# Autodesk Inventor assembly: IntakeAssembly-ver1-1111-2020
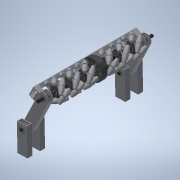
[picture p0: Inventor's stored thumbnail of the model, 180x180]
Saved by Autodesk Inventor 2021 (Build 250183000, 183)
## iProperties
Created: 2020-01-11
Part Number: IntakeAssembly-ver1-1111-2020
Document SubType Name: Assembly
Designer: Power Hawks CADD
Author: Power Hawks CADD
## Documents named in this file (14)
- E:\PHRC CADD 2021\PHRC CADD\2020 Infinite Recharge\Intake\Assemblies\IntakeAssembly-ver1-1111-2020.iam
- E:\PHRC CADD 2021\PHRC CADD\2020 Infinite Recharge\Intake\Parts\0.5inThunderHexShaft-1111-2020.ipt
- E:\PHRC CADD 2021\PHRC CADD\2020 Infinite Recharge\Intake\Parts\Mechanum Wheel.iam
- E:\PHRC CADD 2021\PHRC CADD\2020 Infinite Recharge\Intake\Parts\0.5inAcetalSpacer-1111-2020.ipt
- E:\PHRC CADD 2021\PHRC CADD\Resources\VEXpro Resources\Wheels\4 inch\4IN-CompliantWheel-500Hex.iam
- E:\PHRC CADD 2021\PHRC CADD\Resources\VEXpro Resources\Spacers\0.5inAcetalSpace(0.5inHex)-1111-2016.ipt
- E:\PHRC CADD 2021\PHRC CADD\Resources\VEXpro Resources\Wheels\Mecanum Wheels\4_Mecanum_Wheel_Left_217-3644.iam
- E:\PHRC CADD 2021\PHRC CADD\2020 Infinite Recharge\Intake\Parts\WristBarr.ver1-1111-2020.ipt
- E:\PHRC CADD 2021\PHRC CADD\Resources\VEXpro Resources\Bearings\0.5inHexFlangedBearing(1.125inx0.313in)-1111-2016.ipt
- E:\PHRC CADD 2021\PHRC CADD\2020 Infinite Recharge\Intake\Parts\1x2AluminumSpacer.ver1-1111-2020.ipt
- E:\PHRC CADD 2021\PHRC CADD\2020 Infinite Recharge\Intake\Parts\OverheadSupportBar.ver1-1111-2020.ipt
- E:\PHRC CADD 2021\PHRC CADD\2020 Infinite Recharge\Intake\Parts\WristFulcrum.ver-1111-2020.ipt
- E:\PHRC CADD 2021\PHRC CADD\2020 Infinite Recharge\Intake\Parts\0.5inThunderHexShaft4in-1111-2020.ipt
- E:\PHRC CADD 2021\PHRC CADD\Resources\VEXpro Resources\Spacers\0.125inAcetalSpacer(0.5inHex)-1111-2016.ipt
## Components (47 placed, 13 different names)
1. 0.5inThunderHexShaft-1111-2020:1 — Cylindrical:1, Cylindrical:2, Cylindrical:3, Cylindrical:4, Cylindrical:5, Cylindrical:6, Cylindrical:7, Cylindrical:8, Cylindrical:10, Cylindrical:11, Cylindrical:12, Cylindrical:13, Cylindrical:14, Cylindrical:15, Cylindrical:22, Cylindrical:25, Flush:8
2. Mechanum Wheel:1 [sub-assembly] — Cylindrical:3, Mate:6, Mate:14
3. Mechanum Wheel:2 [sub-assembly] — Cylindrical:2, Mate:8, Mate:9
4. Mechanum Wheel:3 [sub-assembly] — Cylindrical:7, Mate:4, Mate:5
5. Mechanum Wheel:4 [sub-assembly] — Cylindrical:5, Mate:2, Mate:3
6. 0.5inAcetalSpacer-1111-2020:1 — Cylindrical:1, Mate:5, Mate:6
7. 0.5inAcetalSpacer-1111-2020:2 — Cylindrical:4, Mate:1, Mate:2
8. 0.5inAcetalSpacer-1111-2020:3 — Cylindrical:6, Mate:3, Mate:4
9. 4IN-CompliantWheel-500Hex:1 [sub-assembly] — Cylindrical:8, Mate:1, Cylindrical:9, Mate:7
10. 0.5inAcetalSpace(0.5inHex)-1111-2016:1 — Cylindrical:9, Mate:7, Mate:8
11. 0.5inAcetalSpace(0.5inHex)-1111-2016:2 — Cylindrical:10, Mate:9, Mate:10
12. 0.5inAcetalSpace(0.5inHex)-1111-2016:3 — Cylindrical:14, Mate:13, Mate:30
13. 0.5inAcetalSpace(0.5inHex)-1111-2016:4 — Cylindrical:12, Mate:11, Mate:12
14. 4_Mecanum_Wheel_Left_217-3644:1 [sub-assembly] — Cylindrical:13, Mate:12, Mate:13
15. 4_Mecanum_Wheel_Left_217-3644:2 [sub-assembly] — Cylindrical:11, Mate:10, Mate:11
16. 0.5inAcetalSpace(0.5inHex)-1111-2016:5 — Cylindrical:15, Mate:14, Mate:31
17. WristBarr.ver1-1111-2020:1 — Cylindrical:20, Mate:18, Cylindrical:21, Mate:19, Flush:2, Mate:25, Flush:3, Mate:26, Cylindrical:26, Mate:29, Rigid:1
18. WristBarr.ver1-1111-2020:2 — Cylindrical:23, Cylindrical:24, Mate:22, Mate:23, Flush:2, Mate:28, Flush:6, Rigid:2, Rigid:3, Flush:8
19. 0.5inHexFlangedBearing(1.125inx0.313in)-1111-2016:1 — Cylindrical:24, Mate:22
20. 0.5inHexFlangedBearing(1.125inx0.313in)-1111-2016:2 — Cylindrical:23, Mate:23, Cylindrical:25, Mate:30
21. 0.5inHexFlangedBearing(1.125inx0.313in)-1111-2016:4 — Cylindrical:20, Mate:18
22. 0.5inHexFlangedBearing(1.125inx0.313in)-1111-2016:8 — Cylindrical:21, Mate:19, Cylindrical:22, Mate:31
23. OverheadSupportBar.ver1-1111-2020:1 — Mate:27, Flush:4, Flush:5, Flush:7
24. 1x2AluminumSpacer.ver1-1111-2020:1 — Mate:25, Flush:3, Mate:26, Mate:27, Flush:4, Flush:5
25. 1x2AluminumSpacer.ver1-1111-2020:2 — Mate:28, Flush:6, Flush:7
26. 0.5inHexFlangedBearing(1.125inx0.313in)-1111-2016:9 — Rigid:2, Mate:36
27. 0.5inHexFlangedBearing(1.125inx0.313in)-1111-2016:10 — Cylindrical:26, Mate:29, Cylindrical:28, Mate:32
28. 0.5inHexFlangedBearing(1.125inx0.313in)-1111-2016:11 — Rigid:3, Cylindrical:27, Mate:37
29. 0.5inHexFlangedBearing(1.125inx0.313in)-1111-2016:12 — Rigid:1, Mate:34
30. WristFulcrum.ver-1111-2020:1 — Rotational:1, Rotational:2, Flush:9, Flush:10
31. WristFulcrum.ver-1111-2020:2 — Rotational:3, Rotational:4, Flush:9
32. WristFulcrum.ver-1111-2020:3 — Rotational:5, Rotational:6, Flush:10, Flush:11
33. WristFulcrum.ver-1111-2020:4 — Rotational:7, Rotational:8, Flush:11
34. 0.5inHexFlangedBearing(1.125inx0.313in)-1111-2016:13 — Rotational:1, Cylindrical:30, Mate:35
35. 0.5inHexFlangedBearing(1.125inx0.313in)-1111-2016:14 — Rotational:4, Cylindrical:29, Mate:33
36. 0.5inHexFlangedBearing(1.125inx0.313in)-1111-2016:15 — Rotational:2
37. 0.5inHexFlangedBearing(1.125inx0.313in)-1111-2016:16 — Rotational:3, Flush:12
38. 0.5inHexFlangedBearing(1.125inx0.313in)-1111-2016:17 — Rotational:6, Flush:13
39. 0.5inHexFlangedBearing(1.125inx0.313in)-1111-2016:18 — Rotational:8
40. 0.5inHexFlangedBearing(1.125inx0.313in)-1111-2016:19 — Rotational:5, Cylindrical:32, Mate:38
41. 0.5inHexFlangedBearing(1.125inx0.313in)-1111-2016:20 — Rotational:7, Cylindrical:31, Mate:39
42. 0.5inThunderHexShaft4in-1111-2020:1 — Cylindrical:28, Cylindrical:29, Cylindrical:30, Cylindrical:33, Cylindrical:34, Flush:12
43. 0.5inThunderHexShaft4in-1111-2020:2 — Cylindrical:27, Cylindrical:31, Cylindrical:32, Cylindrical:35, Cylindrical:36, Flush:13
44. 0.125inAcetalSpacer(0.5inHex)-1111-2016:1 — Cylindrical:33, Mate:32, Mate:33
45. 0.125inAcetalSpacer(0.5inHex)-1111-2016:2 — Cylindrical:34, Mate:34, Mate:35
46. 0.125inAcetalSpacer(0.5inHex)-1111-2016:3 — Cylindrical:36, Mate:36, Mate:38
47. 0.125inAcetalSpacer(0.5inHex)-1111-2016:4 — Cylindrical:35, Mate:37, Mate:39
## Relationships (88: Mate 33, CylindricalJoint 32, Flush 12, RevoluteJoint 8, WeldJoint 3)
- Cylindrical:1: 0.5inThunderHexShaft-1111-2020:1 ↔ 0.5inAcetalSpacer-1111-2020:1
- Cylindrical:2: 0.5inThunderHexShaft-1111-2020:1 ↔ Mechanum Wheel:2
- Cylindrical:3: 0.5inThunderHexShaft-1111-2020:1 ↔ Mechanum Wheel:1
- Cylindrical:4: 0.5inThunderHexShaft-1111-2020:1 ↔ 0.5inAcetalSpacer-1111-2020:2
- Cylindrical:5: 0.5inThunderHexShaft-1111-2020:1 ↔ Mechanum Wheel:4
- Cylindrical:6: 0.5inThunderHexShaft-1111-2020:1 ↔ 0.5inAcetalSpacer-1111-2020:3
- Cylindrical:7: 0.5inThunderHexShaft-1111-2020:1 ↔ Mechanum Wheel:3
- Cylindrical:8: 0.5inThunderHexShaft-1111-2020:1 ↔ 4IN-CompliantWheel-500Hex:1
- Mate:1: 0.5inAcetalSpacer-1111-2020:2 ↔ 4IN-CompliantWheel-500Hex:1
- Mate:2: Mechanum Wheel:4 ↔ 0.5inAcetalSpacer-1111-2020:2
- Mate:3: Mechanum Wheel:4 ↔ 0.5inAcetalSpacer-1111-2020:3
- Mate:4: Mechanum Wheel:3 ↔ 0.5inAcetalSpacer-1111-2020:3
- Mate:5: Mechanum Wheel:3 ↔ 0.5inAcetalSpacer-1111-2020:1
- Mate:6: Mechanum Wheel:1 ↔ 0.5inAcetalSpacer-1111-2020:1
- Cylindrical:9: 4IN-CompliantWheel-500Hex:1 ↔ 0.5inAcetalSpace(0.5inHex)-1111-2016:1
- Mate:7: 4IN-CompliantWheel-500Hex:1 ↔ 0.5inAcetalSpace(0.5inHex)-1111-2016:1
- Mate:8: Mechanum Wheel:2 ↔ 0.5inAcetalSpace(0.5inHex)-1111-2016:1
- Cylindrical:10: 0.5inThunderHexShaft-1111-2020:1 ↔ 0.5inAcetalSpace(0.5inHex)-1111-2016:2
- Mate:9: Mechanum Wheel:2 ↔ 0.5inAcetalSpace(0.5inHex)-1111-2016:2
- Cylindrical:11: 0.5inThunderHexShaft-1111-2020:1 ↔ 4_Mecanum_Wheel_Left_217-3644:2
- Mate:10: 0.5inAcetalSpace(0.5inHex)-1111-2016:2 ↔ 4_Mecanum_Wheel_Left_217-3644:2
- Cylindrical:12: 0.5inThunderHexShaft-1111-2020:1 ↔ 0.5inAcetalSpace(0.5inHex)-1111-2016:4
- Mate:11: 0.5inAcetalSpace(0.5inHex)-1111-2016:4 ↔ 4_Mecanum_Wheel_Left_217-3644:2
- Cylindrical:13: 0.5inThunderHexShaft-1111-2020:1 ↔ 4_Mecanum_Wheel_Left_217-3644:1
- Mate:12: 0.5inAcetalSpace(0.5inHex)-1111-2016:4 ↔ 4_Mecanum_Wheel_Left_217-3644:1
- Cylindrical:14: 0.5inThunderHexShaft-1111-2020:1 ↔ 0.5inAcetalSpace(0.5inHex)-1111-2016:3
- Mate:13: 0.5inAcetalSpace(0.5inHex)-1111-2016:3 ↔ 4_Mecanum_Wheel_Left_217-3644:1
- Cylindrical:15: 0.5inThunderHexShaft-1111-2020:1 ↔ 0.5inAcetalSpace(0.5inHex)-1111-2016:5
- Mate:14: Mechanum Wheel:1 ↔ 0.5inAcetalSpace(0.5inHex)-1111-2016:5
- Cylindrical:20: WristBarr.ver1-1111-2020:1 ↔ 0.5inHexFlangedBearing(1.125inx0.313in)-1111-2016:4
- Mate:18: WristBarr.ver1-1111-2020:1 ↔ 0.5inHexFlangedBearing(1.125inx0.313in)-1111-2016:4
- Cylindrical:21: WristBarr.ver1-1111-2020:1 ↔ 0.5inHexFlangedBearing(1.125inx0.313in)-1111-2016:8
- Mate:19: WristBarr.ver1-1111-2020:1 ↔ 0.5inHexFlangedBearing(1.125inx0.313in)-1111-2016:8
- Cylindrical:22: 0.5inThunderHexShaft-1111-2020:1 ↔ 0.5inHexFlangedBearing(1.125inx0.313in)-1111-2016:8
- Cylindrical:23: WristBarr.ver1-1111-2020:2 ↔ 0.5inHexFlangedBearing(1.125inx0.313in)-1111-2016:2
- Cylindrical:24: WristBarr.ver1-1111-2020:2 ↔ 0.5inHexFlangedBearing(1.125inx0.313in)-1111-2016:1
- Mate:22: WristBarr.ver1-1111-2020:2 ↔ 0.5inHexFlangedBearing(1.125inx0.313in)-1111-2016:1
- Mate:23: WristBarr.ver1-1111-2020:2 ↔ 0.5inHexFlangedBearing(1.125inx0.313in)-1111-2016:2
- Cylindrical:25: 0.5inThunderHexShaft-1111-2020:1 ↔ 0.5inHexFlangedBearing(1.125inx0.313in)-1111-2016:2
- Flush:2: WristBarr.ver1-1111-2020:1 ↔ WristBarr.ver1-1111-2020:2
- Mate:25: WristBarr.ver1-1111-2020:1 ↔ 1x2AluminumSpacer.ver1-1111-2020:1
- Flush:3: WristBarr.ver1-1111-2020:1 ↔ 1x2AluminumSpacer.ver1-1111-2020:1
- Mate:26: WristBarr.ver1-1111-2020:1 ↔ 1x2AluminumSpacer.ver1-1111-2020:1
- Mate:27: OverheadSupportBar.ver1-1111-2020:1 ↔ 1x2AluminumSpacer.ver1-1111-2020:1
- Flush:4: OverheadSupportBar.ver1-1111-2020:1 ↔ 1x2AluminumSpacer.ver1-1111-2020:1
- Flush:5: OverheadSupportBar.ver1-1111-2020:1 ↔ 1x2AluminumSpacer.ver1-1111-2020:1
- Mate:28: WristBarr.ver1-1111-2020:2 ↔ 1x2AluminumSpacer.ver1-1111-2020:2
- Flush:6: WristBarr.ver1-1111-2020:2 ↔ 1x2AluminumSpacer.ver1-1111-2020:2
- Flush:7: OverheadSupportBar.ver1-1111-2020:1 ↔ 1x2AluminumSpacer.ver1-1111-2020:2
- Cylindrical:26: WristBarr.ver1-1111-2020:1 ↔ 0.5inHexFlangedBearing(1.125inx0.313in)-1111-2016:10
- Mate:29: WristBarr.ver1-1111-2020:1 ↔ 0.5inHexFlangedBearing(1.125inx0.313in)-1111-2016:10
- Rigid:1 [WeldJoint]: WristBarr.ver1-1111-2020:1 ↔ 0.5inHexFlangedBearing(1.125inx0.313in)-1111-2016:12
- Rigid:2 [WeldJoint]: WristBarr.ver1-1111-2020:2 ↔ 0.5inHexFlangedBearing(1.125inx0.313in)-1111-2016:9
- Rigid:3 [WeldJoint]: WristBarr.ver1-1111-2020:2 ↔ 0.5inHexFlangedBearing(1.125inx0.313in)-1111-2016:11
- Mate:30: 0.5inAcetalSpace(0.5inHex)-1111-2016:3 ↔ 0.5inHexFlangedBearing(1.125inx0.313in)-1111-2016:2
- Mate:31: 0.5inAcetalSpace(0.5inHex)-1111-2016:5 ↔ 0.5inHexFlangedBearing(1.125inx0.313in)-1111-2016:8
- Flush:8 (30.1625 mm): 0.5inThunderHexShaft-1111-2020:1 ↔ WristBarr.ver1-1111-2020:2
- Rotational:1 [RevoluteJoint]: WristFulcrum.ver-1111-2020:1 ↔ 0.5inHexFlangedBearing(1.125inx0.313in)-1111-2016:13
- Rotational:2 [RevoluteJoint]: WristFulcrum.ver-1111-2020:1 ↔ 0.5inHexFlangedBearing(1.125inx0.313in)-1111-2016:15
- Rotational:3 [RevoluteJoint]: WristFulcrum.ver-1111-2020:2 ↔ 0.5inHexFlangedBearing(1.125inx0.313in)-1111-2016:16
- Rotational:4 [RevoluteJoint]: WristFulcrum.ver-1111-2020:2 ↔ 0.5inHexFlangedBearing(1.125inx0.313in)-1111-2016:14
- Rotational:5 [RevoluteJoint]: WristFulcrum.ver-1111-2020:3 ↔ 0.5inHexFlangedBearing(1.125inx0.313in)-1111-2016:19
- Rotational:6 [RevoluteJoint]: WristFulcrum.ver-1111-2020:3 ↔ 0.5inHexFlangedBearing(1.125inx0.313in)-1111-2016:17
- Rotational:7 [RevoluteJoint]: WristFulcrum.ver-1111-2020:4 ↔ 0.5inHexFlangedBearing(1.125inx0.313in)-1111-2016:20
- Rotational:8 [RevoluteJoint]: WristFulcrum.ver-1111-2020:4 ↔ 0.5inHexFlangedBearing(1.125inx0.313in)-1111-2016:18
- Cylindrical:27: 0.5inHexFlangedBearing(1.125inx0.313in)-1111-2016:11 ↔ 0.5inThunderHexShaft4in-1111-2020:2
- Cylindrical:28: 0.5inHexFlangedBearing(1.125inx0.313in)-1111-2016:10 ↔ 0.5inThunderHexShaft4in-1111-2020:1
- Cylindrical:29: 0.5inHexFlangedBearing(1.125inx0.313in)-1111-2016:14 ↔ 0.5inThunderHexShaft4in-1111-2020:1
- Cylindrical:30: 0.5inHexFlangedBearing(1.125inx0.313in)-1111-2016:13 ↔ 0.5inThunderHexShaft4in-1111-2020:1
- Cylindrical:31: 0.5inHexFlangedBearing(1.125inx0.313in)-1111-2016:20 ↔ 0.5inThunderHexShaft4in-1111-2020:2
- Cylindrical:32: 0.5inHexFlangedBearing(1.125inx0.313in)-1111-2016:19 ↔ 0.5inThunderHexShaft4in-1111-2020:2
- Flush:9: WristFulcrum.ver-1111-2020:1 ↔ WristFulcrum.ver-1111-2020:2
- Flush:10: WristFulcrum.ver-1111-2020:1 ↔ WristFulcrum.ver-1111-2020:3
- Flush:11: WristFulcrum.ver-1111-2020:3 ↔ WristFulcrum.ver-1111-2020:4
- Cylindrical:33: 0.5inThunderHexShaft4in-1111-2020:1 ↔ 0.125inAcetalSpacer(0.5inHex)-1111-2016:1
- Cylindrical:34: 0.5inThunderHexShaft4in-1111-2020:1 ↔ 0.125inAcetalSpacer(0.5inHex)-1111-2016:2
- Mate:32: 0.5inHexFlangedBearing(1.125inx0.313in)-1111-2016:10 ↔ 0.125inAcetalSpacer(0.5inHex)-1111-2016:1
- Mate:33: 0.5inHexFlangedBearing(1.125inx0.313in)-1111-2016:14 ↔ 0.125inAcetalSpacer(0.5inHex)-1111-2016:1
- Mate:34: 0.5inHexFlangedBearing(1.125inx0.313in)-1111-2016:12 ↔ 0.125inAcetalSpacer(0.5inHex)-1111-2016:2
- Mate:35: 0.5inHexFlangedBearing(1.125inx0.313in)-1111-2016:13 ↔ 0.125inAcetalSpacer(0.5inHex)-1111-2016:2
- Flush:12 (4.3815 mm): 0.5inHexFlangedBearing(1.125inx0.313in)-1111-2016:16 ↔ 0.5inThunderHexShaft4in-1111-2020:1
- Cylindrical:35: 0.5inThunderHexShaft4in-1111-2020:2 ↔ 0.125inAcetalSpacer(0.5inHex)-1111-2016:4
- Cylindrical:36: 0.5inThunderHexShaft4in-1111-2020:2 ↔ 0.125inAcetalSpacer(0.5inHex)-1111-2016:3
- Mate:36: 0.5inHexFlangedBearing(1.125inx0.313in)-1111-2016:9 ↔ 0.125inAcetalSpacer(0.5inHex)-1111-2016:3
- Mate:37: 0.5inHexFlangedBearing(1.125inx0.313in)-1111-2016:11 ↔ 0.125inAcetalSpacer(0.5inHex)-1111-2016:4
- Mate:38: 0.5inHexFlangedBearing(1.125inx0.313in)-1111-2016:19 ↔ 0.125inAcetalSpacer(0.5inHex)-1111-2016:3
- Mate:39: 0.5inHexFlangedBearing(1.125inx0.313in)-1111-2016:20 ↔ 0.125inAcetalSpacer(0.5inHex)-1111-2016:4
- Flush:13 (4.3815 mm): 0.5inHexFlangedBearing(1.125inx0.313in)-1111-2016:17 ↔ 0.5inThunderHexShaft4in-1111-2020:2
